# Autodesk Inventor assembly: VP TRAY PNL PUSHER
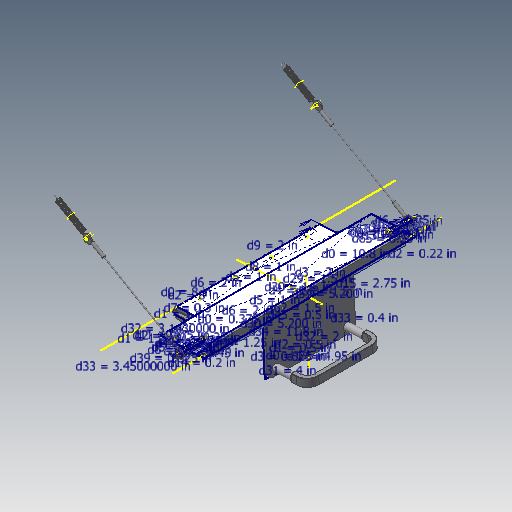
[picture p0: Inventor's stored thumbnail of the model, 512x512]
Saved by Autodesk Inventor 2020.3 (Build 243373000, 373)
## iProperties
RuleStatus: InUse
AfterDocSave0: file://Part Number Cleaner
Created: 2019-10-29
Vendor: HHMI: JRC - ID&F
Document SubType Name: Assembly
Designer: arnoldj
DESIGN DEPARTMENT: HHMI: JRC - ID&F
ALTERED ITEM PART NUMBER: N/A
ALTERED ITEM VENDOR: N/A
ALTERED ITEM DESCRIPTION: N/A
Author: arnoldj
Revision Number: 0
## Documents named in this file (14)
- C:\_WORKSPACE\DATA\PROJECTS\_PROJECTS BY LAB\FLY FACILITY\FLY MEDIA VIAL PLUGGING\VP TRAY PNL PUSHER.iam
- C:\_WORKSPACE\DATA\PROJECTS\_PROJECTS BY LAB\FLY FACILITY\FLY MEDIA VIAL PLUGGING\VP MCMASTER 1569A978 AI .iam
- C:\_WORKSPACE\DATA\PROJECTS\_PROJECTS BY LAB\FLY FACILITY\FLY MEDIA VIAL PLUGGING\VP HINGE SHIFT PLATE.ipt
- C:\_WORKSPACE\DATA\COMMON\Servocity\585600.ipt
- C:\_WORKSPACE\DATA\PROJECTS\_PROJECTS BY LAB\FLY FACILITY\FLY MEDIA VIAL PLUGGING\VP TRAY PUSHER TOP.ipt
- C:\_WORKSPACE\DATA\COMMON\McMaster\MCMASTER 1855A640_PULL HANDLE.ipt
- C:\_WORKSPACE\DATA\PROJECTS\_PROJECTS BY LAB\FLY FACILITY\FLY MEDIA VIAL PLUGGING\VP PUSHER DETENT.ipt
- C:\_WORKSPACE\DATA\PROJECTS\_PROJECTS BY LAB\FLY FACILITY\FLY MEDIA VIAL PLUGGING\VP TRAY PUSHER PNL V2.ipt
- C:\_WORKSPACE\DATA\COMMON\McMaster\MCMASTER 92510A629 1L 8-32 SPACER AL .ipt
- C:\_WORKSPACE\DATA\COMMON\WB JONES\WB JONES_248_Steel Extension Spring.ipt
- C:\_WORKSPACE\DATA\PROJECTS\_PROJECTS BY LAB\FLY FACILITY\FLY MEDIA VIAL PLUGGING\VP SPRING HOLDER.ipt
- C:\_WORKSPACE\DATA\COMMON\McMaster\MCMASTER 30345T138.ipt
- C:\_WORKSPACE\DATA\COMMON\McMaster\MCMASTER 92196A194.ipt
- C:\_WORKSPACE\DATA\COMMON\McMaster\MCMASTER 92141A009.ipt
## Components (23 placed, 13 different names)
1. VP MCMASTER 1569A978 AI :1 [sub-assembly] — Mate:1, Mate:2, Mate:3, Mate:4, Mate:5, Mate:6
2. VP TRAY PUSHER PNL V2:1 — Mate:1, Mate:2, Mate:3, Mate:7, Mate:8, Mate:9, Angle:1, Mate:10, Angle:2, Mate:11, Mate:12, Angle:3, Mate:16, Mate:17, Angle:4, Mate:18, Mate:19, Angle:5, Mate:28, Mate:45, Mate:46, Mate:47, Mate:48, Mate:49, Mate:50
3. VP HINGE SHIFT PLATE:1 — Mate:4, Mate:5, Mate:6
4. 585600:1 — Mate:7, Mate:10, Angle:2, Mate:15
5. 585600:2 — Mate:8, Mate:9, Angle:1, Mate:13, Mate:14
6. 585600:3 — Mate:11, Mate:12, Angle:3
7. VP TRAY PUSHER TOP:1 — Mate:13, Mate:14, Mate:15, Mate:20, Mate:21, Mate:22, Mate:23, Mate:24, Mate:25, Mate:35, Mate:36, Mate:37, Mate:38
8. 585600:4 — Mate:16, Mate:17, Angle:4, Mate:28
9. 585600:5 — Mate:18, Mate:19, Angle:5
10. MCMASTER 1855A640_PULL HANDLE:1 — Mate:20, Mate:21, Mate:22
11. VP PUSHER DETENT:1 — Mate:23, Mate:24, Mate:25
12. MCMASTER 92510A629 1L 8-32 SPACER AL :1 — Mate:35, Mate:38
13. MCMASTER 92510A629 1L 8-32 SPACER AL :2 — Mate:36, Mate:37
14. WB JONES_248_Steel Extension Spring:1 — Mate:53, Mate:54, Angle:6
15. WB JONES_248_Steel Extension Spring:2 — Mate:57, Mate:58, Angle:6
16. VP SPRING HOLDER:1 — Mate:45, Mate:46, Mate:47, Mate:55, Mate:56, Mate:59, Mate:60
17. VP SPRING HOLDER:2 — Mate:48, Mate:49, Mate:50, Mate:51, Mate:52, Mate:63, Mate:64
18. MCMASTER 30345T138:1 — Mate:51, Mate:52, Mate:53, Mate:54, Mate:65
19. MCMASTER 30345T138:2 — Mate:55, Mate:56, Mate:57, Mate:58, Mate:61
20. MCMASTER 92196A194:1 — Mate:63, Mate:64, Mate:66
21. MCMASTER 92196A194:2 — Mate:59, Mate:60, Mate:62
22. MCMASTER 92141A009:1 — Mate:61, Mate:62
23. MCMASTER 92141A009:2 — Mate:65, Mate:66
## Relationships (58: Mate 52, Angle 6)
- Mate:1: VP MCMASTER 1569A978 AI :1 ↔ VP TRAY PUSHER PNL V2:1
- Mate:2: VP MCMASTER 1569A978 AI :1 ↔ VP TRAY PUSHER PNL V2:1
- Mate:3: VP MCMASTER 1569A978 AI :1 ↔ VP TRAY PUSHER PNL V2:1
- Mate:4: VP MCMASTER 1569A978 AI :1 ↔ VP HINGE SHIFT PLATE:1
- Mate:5: VP MCMASTER 1569A978 AI :1 ↔ VP HINGE SHIFT PLATE:1
- Mate:6: VP MCMASTER 1569A978 AI :1 ↔ VP HINGE SHIFT PLATE:1
- Mate:7: VP TRAY PUSHER PNL V2:1 ↔ 585600:1
- Mate:8: VP TRAY PUSHER PNL V2:1 ↔ 585600:2
- Mate:9: VP TRAY PUSHER PNL V2:1 ↔ 585600:2
- Angle:1 (0 deg): VP TRAY PUSHER PNL V2:1 ↔ 585600:2
- Mate:10: VP TRAY PUSHER PNL V2:1 ↔ 585600:1
- Angle:2 (0 deg): VP TRAY PUSHER PNL V2:1 ↔ 585600:1
- Mate:11: VP TRAY PUSHER PNL V2:1 ↔ 585600:3
- Mate:12: VP TRAY PUSHER PNL V2:1 ↔ 585600:3
- Angle:3 (0 deg): VP TRAY PUSHER PNL V2:1 ↔ 585600:3
- Mate:13: 585600:2 ↔ VP TRAY PUSHER TOP:1
- Mate:14: 585600:2 ↔ VP TRAY PUSHER TOP:1
- Mate:15: 585600:1 ↔ VP TRAY PUSHER TOP:1
- Mate:16: VP TRAY PUSHER PNL V2:1 ↔ 585600:4
- Mate:17: VP TRAY PUSHER PNL V2:1 ↔ 585600:4
- Angle:4 (0 deg): VP TRAY PUSHER PNL V2:1 ↔ 585600:4
- Mate:18: VP TRAY PUSHER PNL V2:1 ↔ 585600:5
- Mate:19: VP TRAY PUSHER PNL V2:1 ↔ 585600:5
- Angle:5 (0 deg): VP TRAY PUSHER PNL V2:1 ↔ 585600:5
- Mate:20 (25.4 mm): VP TRAY PUSHER TOP:1 ↔ MCMASTER 1855A640_PULL HANDLE:1
- Mate:21: VP TRAY PUSHER TOP:1 ↔ MCMASTER 1855A640_PULL HANDLE:1
- Mate:22: VP TRAY PUSHER TOP:1 ↔ MCMASTER 1855A640_PULL HANDLE:1
- Mate:23: VP TRAY PUSHER TOP:1 ↔ VP PUSHER DETENT:1
- Mate:24: VP TRAY PUSHER TOP:1 ↔ VP PUSHER DETENT:1
- Mate:25: VP TRAY PUSHER TOP:1 ↔ VP PUSHER DETENT:1
- Mate:28: VP TRAY PUSHER PNL V2:1 ↔ 585600:4
- Mate:35: VP TRAY PUSHER TOP:1 ↔ MCMASTER 92510A629 1L 8-32 SPACER AL :1
- Mate:36: VP TRAY PUSHER TOP:1 ↔ MCMASTER 92510A629 1L 8-32 SPACER AL :2
- Mate:37: VP TRAY PUSHER TOP:1 ↔ MCMASTER 92510A629 1L 8-32 SPACER AL :2
- Mate:38: VP TRAY PUSHER TOP:1 ↔ MCMASTER 92510A629 1L 8-32 SPACER AL :1
- Mate:45: VP TRAY PUSHER PNL V2:1 ↔ VP SPRING HOLDER:1
- Mate:46: VP TRAY PUSHER PNL V2:1 ↔ VP SPRING HOLDER:1
- Mate:47: VP TRAY PUSHER PNL V2:1 ↔ VP SPRING HOLDER:1
- Mate:48: VP TRAY PUSHER PNL V2:1 ↔ VP SPRING HOLDER:2
- Mate:49: VP TRAY PUSHER PNL V2:1 ↔ VP SPRING HOLDER:2
- Mate:50: VP TRAY PUSHER PNL V2:1 ↔ VP SPRING HOLDER:2
- Mate:51 (0.508 mm): VP SPRING HOLDER:2 ↔ MCMASTER 30345T138:1
- Mate:52: VP SPRING HOLDER:2 ↔ MCMASTER 30345T138:1
- Mate:53: WB JONES_248_Steel Extension Spring:1 ↔ MCMASTER 30345T138:1
- Mate:54 (1.905 mm): WB JONES_248_Steel Extension Spring:1 ↔ MCMASTER 30345T138:1
- Mate:55 (0.508 mm): VP SPRING HOLDER:1 ↔ MCMASTER 30345T138:2
- Mate:56: VP SPRING HOLDER:1 ↔ MCMASTER 30345T138:2
- Mate:57: WB JONES_248_Steel Extension Spring:2 ↔ MCMASTER 30345T138:2
- Mate:58 (1.905 mm): WB JONES_248_Steel Extension Spring:2 ↔ MCMASTER 30345T138:2
- Angle:6 (0 deg): WB JONES_248_Steel Extension Spring:1 ↔ WB JONES_248_Steel Extension Spring:2
- Mate:59 (-8.89 mm): VP SPRING HOLDER:1 ↔ MCMASTER 92196A194:2
- Mate:60: VP SPRING HOLDER:1 ↔ MCMASTER 92196A194:2
- Mate:61: MCMASTER 30345T138:2 ↔ MCMASTER 92141A009:1
- Mate:62: MCMASTER 92196A194:2 ↔ MCMASTER 92141A009:1
- Mate:63 (-8.89 mm): VP SPRING HOLDER:2 ↔ MCMASTER 92196A194:1
- Mate:64: VP SPRING HOLDER:2 ↔ MCMASTER 92196A194:1
- Mate:65: MCMASTER 30345T138:1 ↔ MCMASTER 92141A009:2
- Mate:66: MCMASTER 92196A194:1 ↔ MCMASTER 92141A009:2
